# Autodesk Inventor assembly: Sketch Heaven
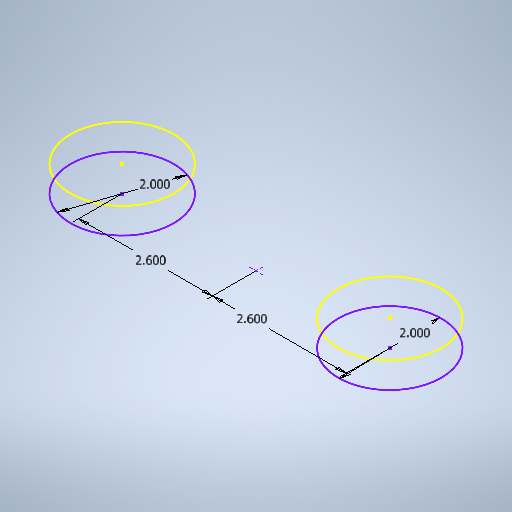
[picture p0: Inventor's stored thumbnail of the model, 512x512]
Saved by Autodesk Inventor 2025.2 (Build 292293000, 293)
## iProperties
Created: 2025-07-21
Part Number: Sketch Heaven
Document SubType Name: Assembly
Designer: Jahan
Author: Jahan
## Documents named in this file (1)
- C:\3284b-cad-2025\Robots\Highlander\Sketch Heaven.iam
## Relationships (1: Flush 1)
- Flush:1 (12.7 mm)
